# Autodesk Inventor assembly: 部件1
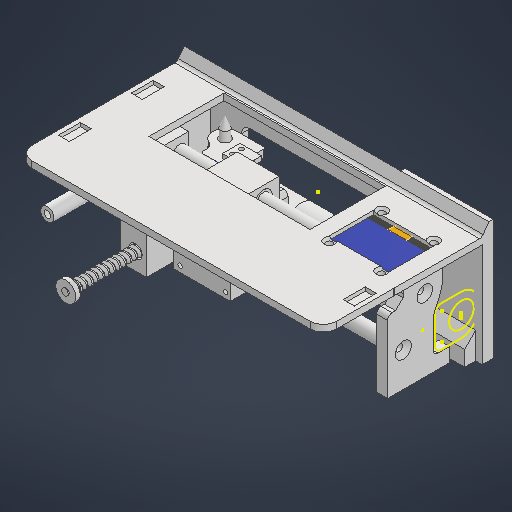
[picture p0: Inventor's stored thumbnail of the model, 512x512]
Saved by Autodesk Inventor 2025 (Build 290162000, 162)
## iProperties
Created: 2025-11-30
Part Number: 部件1
Document SubType Name: Assembly
Designer: XH
Author: XH
## Documents named in this file (18)
- C:\1A_Engineering_files\braille-printer-v2\部件1.iam
- C:\1A_Engineering_files\braille-printer-v2\便签.ipt
- C:\1A_Engineering_files\braille-printer-v2\主体.ipt
- C:\1A_Engineering_files\braille-printer-v2\针头主体.iam
- C:\1A_Engineering_files\braille-printer-v2\钢轴.ipt
- C:\1A_Engineering_files\braille-printer-v2\Y轴杠轴.ipt
- C:\1A_Engineering_files\braille-printer-v2\xy转接连杆.ipt
- C:\1A_Engineering_files\braille-printer-v2\阻挡X轴.ipt
- C:\1A_Engineering_files\braille-printer-v2\大外壳.ipt
- C:\1A_Engineering_files\braille-printer-v2\电机.ipt
- C:\1A_Engineering_files\braille-printer-v2\后盖电路.ipt
- C:\1A_Engineering_files\braille-printer-v2\前舵机位置控制.ipt
- C:\1A_Engineering_files\braille-printer-v2\Weewooday I2C OLED 0.96'' 128x64.iam
- C:\1A_Engineering_files\braille-printer-v2\磁铁.ipt
- C:\1A_Engineering_files\braille-printer-v2\丝杆.ipt
- C:\Users\XH\Documents\Inventor\Content Center Files\R2025\zh-CN\AS 1420\AS 1420 - 1973 - M3 x 8.ipt
- C:\1A_Engineering_files\braille-printer-v2\滚珠轴承.ipt
- C:\1A_Engineering_files\braille-printer-v2\皮带.ipt
## Components (22 placed, 17 different names)
1. 便签:1 — 配合:1, 配合:2
2. 主体:1 — 配合:1, 配合:2, 表面齐平:7, 配合:12, 配合:19, 表面齐平:10, 表面齐平:11, 配合:23, 配合:26, 表面齐平:12, 表面齐平:13, 配合:27, 配合:28, 配合:29, 配合:30, 配合:31, 配合:32, 配合:49, 配合:50
3. 针头主体:1 [sub-assembly] — 配合:5, 配合:34, 配合:51
4. 钢轴:2 — 配合:5, 配合:38, 表面齐平:14, 配合:47
5. Y轴杠轴:2 — 配合:12, 配合:36, 配合:50
6. xy转接连杆:1 — 表面齐平:7, 配合:22, 配合:36, 配合:37, 配合:38, 配合:40, 配合:41, 配合:42, 配合:43
7. 阻挡X轴:1 — 配合:45, 配合:46, 配合:47
8. 大外壳:1 — 配合:19, 表面齐平:10, 表面齐平:11, 配合:25
9. 电机:1 — 配合:22, 配合:23, 配合:33
10. 后盖电路:1 — 配合:25
11. 前舵机位置控制:1 — 配合:26, 表面齐平:12, 表面齐平:13
12. Weewooday I2C OLED 0.96'' 128x64:1 [sub-assembly] — 配合:27, 配合:28, 配合:29
13. 磁铁:1 — 配合:30
14. 磁铁:2 — 配合:31
15. 磁铁:3 — 配合:32
16. 丝杆:1 — 配合:33, 配合:48
17. 钢轴:3 — 配合:34, 配合:37, 表面齐平:14, 配合:43, 配合:45, 配合:46
18. AS 1420 - 公制 M3 x 8:1 — 配合:40, 配合:42
19. AS 1420 - 公制 M3 x 8:2 — 配合:41
20. 滚珠轴承:1 — 配合:48
21. AS 1420 - 公制 M3 x 8:3 — 配合:49
22. 皮带:1 — 配合:51
## Relationships (37: Mate 31, Flush 6)
- 配合:1 [Mate]: 便签:1 ↔ 主体:1
- 配合:2 [Mate]: 便签:1 ↔ 主体:1
- 配合:5 [Mate]: 针头主体:1 ↔ 钢轴:2
- 表面齐平:7 [Flush]: 主体:1 ↔ xy转接连杆:1
- 配合:12 [Mate]: 主体:1 ↔ Y轴杠轴:2
- 配合:19 [Mate]: 主体:1 ↔ 大外壳:1
- 表面齐平:10 [Flush]: 主体:1 ↔ 大外壳:1
- 表面齐平:11 [Flush]: 主体:1 ↔ 大外壳:1
- 配合:22 [Mate]: xy转接连杆:1 ↔ 电机:1
- 配合:23 [Mate]: 主体:1 ↔ 电机:1
- 配合:25 [Mate]: 大外壳:1 ↔ 后盖电路:1
- 配合:26 [Mate]: 主体:1 ↔ 前舵机位置控制:1
- 表面齐平:12 [Flush]: 主体:1 ↔ 前舵机位置控制:1
- 表面齐平:13 [Flush]: 主体:1 ↔ 前舵机位置控制:1
- 配合:27 [Mate]: 主体:1 ↔ Weewooday I2C OLED 0.96'' 128x64:1
- 配合:28 [Mate]: 主体:1 ↔ Weewooday I2C OLED 0.96'' 128x64:1
- 配合:29 [Mate]: 主体:1 ↔ Weewooday I2C OLED 0.96'' 128x64:1
- 配合:30 [Mate]: 主体:1 ↔ 磁铁:1
- 配合:31 [Mate]: 主体:1 ↔ 磁铁:2
- 配合:32 [Mate]: 主体:1 ↔ 磁铁:3
- 配合:33 [Mate]: 电机:1 ↔ 丝杆:1
- 配合:34 [Mate]: 针头主体:1 ↔ 钢轴:3
- 配合:36 [Mate]: Y轴杠轴:2 ↔ xy转接连杆:1
- 配合:37 [Mate]: xy转接连杆:1 ↔ 钢轴:3
- 配合:38 [Mate]: 钢轴:2 ↔ xy转接连杆:1
- 表面齐平:14 [Flush]: 钢轴:2 ↔ 钢轴:3
- 配合:40 [Mate]: xy转接连杆:1 ↔ AS 1420 - 公制 M3 x 8:1
- 配合:41 [Mate]: xy转接连杆:1 ↔ AS 1420 - 公制 M3 x 8:2
- 配合:42 [Mate]: xy转接连杆:1 ↔ AS 1420 - 公制 M3 x 8:1
- 配合:43 [Mate]: xy转接连杆:1 ↔ 钢轴:3
- 配合:45 [Mate]: 阻挡X轴:1 ↔ 钢轴:3
- 配合:46 [Mate]: 阻挡X轴:1 ↔ 钢轴:3
- 配合:47 [Mate]: 钢轴:2 ↔ 阻挡X轴:1
- 配合:48 [Mate]: 丝杆:1 ↔ 滚珠轴承:1
- 配合:49 [Mate]: 主体:1 ↔ AS 1420 - 公制 M3 x 8:3
- 配合:50 [Mate]: 主体:1 ↔ Y轴杠轴:2
- 配合:51 [Mate]: 针头主体:1 ↔ 皮带:1
